# Autodesk Inventor assembly: Mechanics Assembly
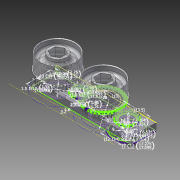
[picture p0: Inventor's stored thumbnail of the model, 180x180]
Saved by Autodesk Inventor 2014 (Build 180170000, 170)
## iProperties
Created: 2013-09-11
Part Number: Mechanics Assembly
Document SubType Name: Assembly
Designer: Brandon
Author: Brandon
## Documents named in this file (7)
- C:\Users\Brandon\Documents\Micromouse\3D\Mechanics Assembly.iam
- C:\Users\Brandon\Documents\Micromouse\3D\Wheel.ipt
- C:\Users\Brandon\Documents\Micromouse\3D\Wheel2Wheel.ipt
- C:\Users\Brandon\Documents\Micromouse\3D\Wheel_MIR.ipt
- C:\Users\Brandon\Documents\Micromouse\3D\mount.ipt
- C:\Users\Brandon\Documents\Micromouse\3D\Mechanics Assembly\Design Accelerator\Spur Gears1.iam
- C:\Users\Brandon\Documents\Micromouse\3D\gear motor.ipt
## Components (6 placed, 6 different names)
1. Wheel:1 — Rotation:3, Mate:4, Rotational:2, Rotation:5
2. Wheel2Wheel:1 — Mate:1, Rotation:3, Mate:2, Mate:5, Rotational:3, Rotation:4
3. Wheel_MIR:1 — Rotational:1, Rotation:4
4. mount:1 — Rotational:1, Rotational:2, Rotational:3, Rotational:4
5. Spur Gears:1 [sub-assembly]
6. gear motor:1 — Rotational:4, Rotation:5
## Relationships (13: Mate 4, RevoluteJoint 4, RelateRotation 3, Angle 1, Flush 1)
- Mate:1: Wheel2Wheel:1
- Rotation:3 [RelateRotation] (0.667 ul): Wheel:1 ↔ Wheel2Wheel:1
- Mate:2: Wheel2Wheel:1
- Angle:1 (0 deg)
- Mate:4 (-1.25 mm): Wheel:1
- Flush:1 (-2.75 mm)
- Mate:5 (-1.5 mm): Wheel2Wheel:1
- Rotational:1 [RevoluteJoint]: Wheel_MIR:1 ↔ mount:1
- Rotational:2 [RevoluteJoint]: Wheel:1 ↔ mount:1
- Rotational:3 [RevoluteJoint] (-1.25 mm): Wheel2Wheel:1 ↔ mount:1
- Rotation:4 [RelateRotation] (1.5 ul): Wheel2Wheel:1 ↔ Wheel_MIR:1
- Rotational:4 [RevoluteJoint] (0.2 mm): mount:1 ↔ gear motor:1
- Rotation:5 [RelateRotation] (2 ul): Wheel:1 ↔ gear motor:1
